# Autodesk Inventor assembly: Test_Button_Assembly
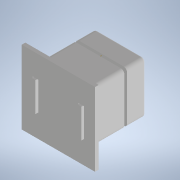
[picture p0: Inventor's stored thumbnail of the model, 180x180]
Saved by Autodesk Inventor 2021 (Build 250183000, 183)
## iProperties
Created: 2020-06-04
Part Number: Test_Button_Assembly
Document SubType Name: Assembly
Designer: ridvansong
Author: ridvansong
## Documents named in this file (5)
- \\Mac\Home\Documents\OP-1 Project\ipt_files\Test_Button_Assembly.iam
- \\Mac\Home\Documents\OP-1 Project\ipt_files\Button Prong.ipt
- \\Mac\Home\Documents\OP-1 Project\ipt_files\Small_Button.ipt
- \\Mac\Home\Documents\OP-1 Project\ipt_files\Small_Button_Base.ipt
- \\Mac\Home\Documents\OP-1 Project\ipt_files\Test_Button_Backboard.ipt
## Components (4 placed, 4 different names)
1. Button Prong:1 — Mate:5, Mate:4, Mate:6, Mate:7
2. Small_Button:1 — Mate:6, Flush:1, Flush:2
3. Small_Button_Base:1 — Mate:1, Mate:2, Mate:3, Mate:5, Mate:4, Flush:1, Flush:2, Mate:7
4. Test_Button_Backboard:1 — Mate:1, Mate:2, Mate:3
## Relationships (9: Mate 7, Flush 2)
- Mate:1: Small_Button_Base:1 ↔ Test_Button_Backboard:1
- Mate:2 (0.25 mm): Small_Button_Base:1 ↔ Test_Button_Backboard:1
- Mate:3: Small_Button_Base:1 ↔ Test_Button_Backboard:1
- Mate:5 (0.5 mm): Button Prong:1 ↔ Small_Button_Base:1
- Mate:4 (0.5 mm): Button Prong:1 ↔ Small_Button_Base:1
- Mate:6: Button Prong:1 ↔ Small_Button:1
- Flush:1: Small_Button:1 ↔ Small_Button_Base:1
- Flush:2: Small_Button:1 ↔ Small_Button_Base:1
- Mate:7: Button Prong:1 ↔ Small_Button_Base:1
